# Autodesk Inventor assembly: Assembly1
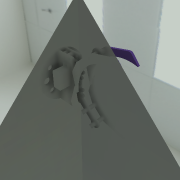
[picture p0: Inventor's stored thumbnail of the model, 180x180]
Saved by Autodesk Inventor 2015 (Build 190159000, 159)
## iProperties
Created: 2015-03-07
Part Number: Assembly1
Document SubType Name: Assembly
Designer: M Sobrun Ibnu Atfal
Author: M Sobrun Ibnu Atfal
## Documents named in this file (11)
- F:\Kegiatan di PENS\proyek robotika\Assembly1.iam
- F:\Kegiatan di PENS\proyek robotika\coba.ipt
- F:\Kegiatan di PENS\proyek robotika\coba3.ipt
- F:\Kegiatan di PENS\proyek robotika\Part1.ipt
- F:\Kegiatan Umum\Sekolah Robot\Robot Rescue\mini_servo.ipt
- F:\Kegiatan di PENS\proyek robotika\Servo_place_grip.ipt
- F:\Kegiatan di PENS\proyek robotika\Servo_place_grip_up.ipt
- F:\Kegiatan di PENS\proyek robotika\spacer8mm.ipt
- F:\Kegiatan di PENS\proyek robotika\spacer12mm.ipt
- F:\Kegiatan di PENS\proyek robotika\penyangga.ipt
- F:\Kegiatan di PENS\proyek robotika\join_w_grandServo.ipt
## Components (23 placed, 10 different names)
1. coba:1 — Insert:11, Insert:25, Insert:26
2. coba3:1 — Insert:14, Insert:35, Insert:36, Insert:38
3. Part1:1 — Insert:33, Insert:34
4. Part1:2 — Insert:31, Insert:32
5. Part1:3 — Insert:27, Insert:28
6. mini_servo:1 — Insert:11, Insert:12, Insert:13
7. Servo_place_grip:1 — Insert:12, Insert:13, Insert:14, Insert:15, Insert:16, Insert:41, Mate:1
8. Servo_place_grip_up:1 — Insert:15, Insert:16, Insert:17, Insert:18, Insert:19, Insert:20, Mate:2, Mate:3
9. spacer8mm:1 — Insert:17
10. spacer8mm:2 — Insert:19
11. spacer8mm:3 — Insert:18
12. spacer8mm:4 — Insert:20
13. spacer8mm:7 — Insert:26, Insert:28, Insert:30
14. spacer8mm:8 — Insert:25, Insert:27, Insert:29
15. spacer8mm:9 — Insert:30, Insert:32
16. spacer8mm:10 — Insert:29, Insert:31
17. spacer12mm:1 — Insert:33, Insert:36
18. spacer12mm:2 — Insert:34, Insert:35, Insert:37
19. spacer12mm:3 — Insert:38, Insert:39
20. spacer12mm:4 — Insert:37, Insert:40
21. Part1:4 — Insert:39, Insert:40
22. penyangga:1 — Insert:41
23. join_w_grandServo:1 — Mate:1, Mate:2, Mate:3
## Relationships (30: Insert 27, Mate 3)
- Insert:11: coba:1 ↔ mini_servo:1
- Insert:12: mini_servo:1 ↔ Servo_place_grip:1
- Insert:13: mini_servo:1 ↔ Servo_place_grip:1
- Insert:14 (5 mm): coba3:1 ↔ Servo_place_grip:1
- Insert:15 (8 mm): Servo_place_grip:1 ↔ Servo_place_grip_up:1
- Insert:16 (8 mm): Servo_place_grip:1 ↔ Servo_place_grip_up:1
- Insert:17: Servo_place_grip_up:1 ↔ spacer8mm:1
- Insert:18: Servo_place_grip_up:1 ↔ spacer8mm:3
- Insert:19: Servo_place_grip_up:1 ↔ spacer8mm:2
- Insert:20: Servo_place_grip_up:1 ↔ spacer8mm:4
- Insert:25: coba:1 ↔ spacer8mm:8
- Insert:26: coba:1 ↔ spacer8mm:7
- Insert:27: Part1:3 ↔ spacer8mm:8
- Insert:28: Part1:3 ↔ spacer8mm:7
- Insert:29: spacer8mm:8 ↔ spacer8mm:10
- Insert:30: spacer8mm:7 ↔ spacer8mm:9
- Insert:31: Part1:2 ↔ spacer8mm:10
- Insert:32: Part1:2 ↔ spacer8mm:9
- Insert:33: Part1:1 ↔ spacer12mm:1
- Insert:34: Part1:1 ↔ spacer12mm:2
- Insert:35: coba3:1 ↔ spacer12mm:2
- Insert:36: coba3:1 ↔ spacer12mm:1
- Insert:37: spacer12mm:2 ↔ spacer12mm:4
- Insert:38: coba3:1 ↔ spacer12mm:3
- Insert:39: spacer12mm:3 ↔ Part1:4
- Insert:40: spacer12mm:4 ↔ Part1:4
- Insert:41: Servo_place_grip:1 ↔ penyangga:1
- Mate:1: Servo_place_grip:1 ↔ join_w_grandServo:1
- Mate:2: Servo_place_grip_up:1 ↔ join_w_grandServo:1
- Mate:3: Servo_place_grip_up:1 ↔ join_w_grandServo:1
